# Autodesk Inventor assembly: CrossBot
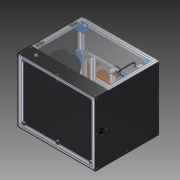
[picture p0: Inventor's stored thumbnail of the model, 180x180]
Saved by Autodesk Inventor 2015 SP1 (Build 190203100, 203)
## iProperties
Created: 2014-08-14
Part Number: CrossBot
Document SubType Name: Assembly
Designer: t_clevj
Mass: 14844.5 g
Surface Area: 49855.2 cm^2
Volume: 9320.22 cm^3
Density: 1.59271 g/cm^3
Author: t_clevj
## Documents named in this file (26)
- C:\Users\Jack\ownCloud\Projects\CrossBot\InventorModel\CrossBot.iam
- C:\Users\Jack\ownCloud\Projects\CrossBot\InventorModel\Frame\Frame.iam
- C:\Users\Jack\ownCloud\Projects\CrossBot\InventorModel\Hardware\Shaft\Shaft8\YShaft.ipt
- C:\Users\Jack\ownCloud\Projects\CrossBot\InventorModel\YAxis\YAxisMotorLeft.iam
- C:\Users\Jack\ownCloud\Projects\CrossBot\InventorModel\YAxis\YAxisIdlerLeft.iam
- C:\Users\Jack\ownCloud\Projects\CrossBot\InventorModel\YAxis\YAxisMotorRight.iam
- C:\Users\Jack\ownCloud\Projects\CrossBot\InventorModel\XAxis\XEndLeft.iam
- C:\Users\Jack\ownCloud\Projects\CrossBot\InventorModel\YAxis\YAxisIdlerRight.iam
- C:\Users\Jack\ownCloud\Projects\CrossBot\InventorModel\XAxis\XEndRight.iam
- C:\Users\Jack\ownCloud\Projects\CrossBot\InventorModel\Hardware\Shaft\Shaft8\XShaft.ipt
- C:\Users\Jack\ownCloud\Projects\CrossBot\InventorModel\Hardware\Shaft\Shaft10\ZAxisShaft.ipt
- C:\Users\Jack\ownCloud\Projects\CrossBot\InventorModel\Enclosure\SpoolFilament.ipt
- C:\Users\Jack\ownCloud\Projects\CrossBot\InventorModel\XAxis\XCarriage.iam
- C:\Users\Jack\ownCloud\Projects\CrossBot\InventorModel\Electronics\PSUUltibots.ipt
- C:\Users\Jack\ownCloud\Projects\CrossBot\InventorModel\Extruder\SanladererBowdenExtruder\SanladererBowdenExtruder.iam
- C:\Users\Jack\ownCloud\Projects\CrossBot\InventorModel\Extruder\SanladererBowdenExtruder\SanladererBowdenExtruderMirrored.iam
- C:\Users\Jack\ownCloud\Projects\CrossBot\InventorModel\ZAxis\ZAxisBed.iam
- C:\Users\Jack\ownCloud\Projects\CrossBot\InventorModel\Electronics\LCD\RepRapDiscountGLCD.ipt
- C:\Users\Jack\ownCloud\Projects\CrossBot\InventorModel\Electronics\Boards\Smoothieboard.ipt
- C:\Users\Jack\ownCloud\Projects\CrossBot\InventorModel\Hardware\Nuts\ExtrusionNuts\ExtrusionNutHNTT5-4.ipt
- C:\Users\Jack\ownCloud\Projects\CrossBot\InventorModel\ZAxis\ZAxisRodClamp.iam
- C:\Users\Jack\ownCloud\Projects\CrossBot\InventorModel\ZAxis\ZDrive.iam
- C:\Users\Jack\ownCloud\Projects\CrossBot\InventorModel\Electronics\KeySwitch\KeySwitch.iam
- C:\Users\Jack\ownCloud\Projects\CrossBot\InventorModel\Electronics\Fans\Fan40x20mm.ipt
- C:\Users\Jack\ownCloud\Projects\CrossBot\InventorModel\ZAxis\ZEndstop.iam
- C:\Users\Jack\ownCloud\Projects\CrossBot\InventorModel\Electronics\Ports\PowerSocket.ipt
## Components (63 placed, 25 different names)
1. Frame:1 [sub-assembly] — Mate:6, Mate:23, Mate:24, Mate:25, Mate:27, Mate:28, Mate:29, Mate:30, Mate:31, Mate:32, Mate:69, Mate:70, Angle:13, Angle:14, Mate:260, Flush:89, Mate:261, Flush:90, Angle:15, Mate:312, Mate:313, Mate:317, Angle:16, Mate:319, Angle:17, Mate:321, Angle:18, Mate:323, Angle:19, Mate:326, Mate:327, Angle:20, Angle:21, Mate:329, Angle:22, Mate:331, Angle:23, Mate:333, Angle:24, Mate:336, Angle:25, Mate:338, Angle:26, Mate:340, Angle:27, Mate:344, Angle:28, Mate:345, Angle:29, Flush:92, Flush:93, Flush:94, Flush:95, Mate:352, Mate:353, Mate:354, Mate:355, Flush:98, Mate:358, Angle:30, Mate:360, Angle:31, Mate:362, Angle:32, Mate:364, Angle:33, Mate:366, Angle:34, Mate:368, Mate:370, Angle:35, Mate:372, Angle:36, Angle:37, Mate:377, Mate:378, Mate:379, Mate:380, Angle:38, Angle:39, Angle:40, Angle:41, Mate:381, Mate:382, Mate:383, Angle:42, Angle:43, Angle:44, Angle:45, Mate:389, Mate:390, Mate:391, Mate:392, Mate:400, Mate:401, Mate:402, Angle:46, Mate:417, Mate:418, Mate:419, Mate:420, Mate:421, Mate:422, Mate:423, Mate:424, Mate:425, Mate:426, Mate:427, Mate:428
2. ZEndstop:1 [sub-assembly] — Mate:415, Angle:46, Mate:416
3. ZDrive:1 [sub-assembly] — Mate:381, Mate:382, Mate:383, Mate:384, Mate:385, Mate:386, Mate:387, Mate:388
4. ExtrusionNutHNTT5-4:29 — Mate:385, Angle:44, Mate:390
5. ExtrusionNutHNTT5-4:30 — Mate:386, Angle:45, Mate:389
6. ExtrusionNutHNTT5-4:31 — Mate:387, Angle:43, Mate:392
7. ExtrusionNutHNTT5-4:32 — Mate:388, Angle:42, Mate:391
8. ExtrusionNutHNTT5-4:16 — Mate:357, Mate:358, Angle:30
9. ExtrusionNutHNTT5-4:17 — Mate:359, Mate:360, Angle:31
10. ExtrusionNutHNTT5-4:18 — Mate:361, Mate:362, Angle:32
11. ExtrusionNutHNTT5-4:19 — Mate:363, Mate:364, Angle:33
12. ExtrusionNutHNTT5-4:20 — Mate:367, Angle:34, Mate:368
13. ExtrusionNutHNTT5-4:21 — Mate:365, Mate:366, Angle:37
14. ExtrusionNutHNTT5-4:22 — Mate:369, Mate:370, Angle:35
15. ExtrusionNutHNTT5-4:24 — Mate:371, Mate:372, Angle:36
16. ZAxisRodClamp:4 [sub-assembly] — Mate:350, Flush:95, Mate:355, Mate:365, Mate:367, Mate:384
17. ZAxisRodClamp:3 [sub-assembly] — Mate:349, Flush:94, Mate:352, Flush:97, Mate:357, Mate:359, Mate:416
18. ZAxisRodClamp:2 [sub-assembly] — Mate:348, Flush:92, Mate:354, Mate:369, Mate:371
19. ZAxisRodClamp:1 [sub-assembly] — Mate:347, Flush:93, Mate:353, Flush:96, Mate:361, Mate:363
20. ZAxisBed:1 [sub-assembly] — Mate:314, Mate:315
21. ZAxisShaft:1 — Mate:315, Mate:349, Mate:350, Mate:351, Flush:97, Mate:415
22. ZAxisShaft:2 — Mate:314, Mate:347, Mate:348, Mate:351, Flush:96
23. YShaft:2 — Mate:26, Mate:124, Mate:130, Mate:187
24. YShaft:3 — Mate:37, Mate:190
25. YAxisMotorLeft:1 [sub-assembly] — Mate:23, Mate:24, Mate:25, Mate:26, Mate:324, Mate:325, Mate:328, Mate:330
26. YAxisMotorRight:1 [sub-assembly] — Mate:30, Mate:31, Mate:32, Mate:37, Mate:316, Mate:318, Mate:320, Mate:322
27. YAxisIdlerLeft:1 [sub-assembly] — Mate:27, Mate:28, Mate:29, Mate:130, Mate:337, Mate:339, Mate:341
28. YAxisIdlerRight:1 [sub-assembly] — Mate:334, Mate:335, Mate:342, Mate:343, Mate:426, Mate:427, Mate:428
29. XShaft:1 — Mate:189, Flush:54, Mate:242
30. XShaft:2 — Mate:188, Flush:55, Mate:191, Mate:241
31. XCarriage:1 [sub-assembly] — Mate:241, Mate:242
32. XEndLeft:1 [sub-assembly] — Mate:124, Mate:187, Mate:188, Mate:189, Flush:54, Flush:55, Angle:14
33. XEndRight:1 [sub-assembly] — Mate:190, Mate:191, Angle:13
34. KeySwitch:1 [sub-assembly] — Mate:400, Mate:401, Mate:402
35. Fan40x20mm:1 — Mate:423, Mate:424, Mate:425
36. Fan40x20mm:3 — Mate:420, Mate:421, Mate:422
37. PowerSocket:1 — Mate:417, Mate:418, Mate:419
38. Smoothieboard:1 — Mate:312
39. RepRapDiscountGLCD:1 — Angle:15
40. PSUUltibots:1 — Mate:313
41. ExtrusionNutHNTT5-4:25 — Mate:373, Mate:380, Angle:38
42. ExtrusionNutHNTT5-4:26 — Mate:374, Mate:378, Angle:39
43. ExtrusionNutHNTT5-4:27 — Mate:375, Mate:379, Angle:40
44. ExtrusionNutHNTT5-4:28 — Mate:376, Mate:377, Angle:41
45. SanladererBowdenExtruderMirrored:1 [sub-assembly] — Mate:261, Flush:90, Flush:91, Mate:373, Mate:376
46. SanladererBowdenExtruder:1 [sub-assembly] — Mate:260, Flush:89, Flush:91, Flush:98, Mate:374, Mate:375
47. SpoolFilament:2 — Mate:309
48. SpoolFilament:1 — Mate:309
49. ExtrusionNutHNTT5-4:1 — Mate:316, Mate:317, Angle:16
50. ExtrusionNutHNTT5-4:2 — Mate:318, Mate:319, Angle:17
51. ExtrusionNutHNTT5-4:3 — Mate:320, Mate:321, Angle:18
52. ExtrusionNutHNTT5-4:4 — Mate:322, Mate:323, Angle:19
53. ExtrusionNutHNTT5-4:5 — Mate:324, Mate:327, Angle:20
54. ExtrusionNutHNTT5-4:6 — Mate:325, Mate:326, Angle:21
55. ExtrusionNutHNTT5-4:7 — Mate:328, Mate:329, Angle:22
56. ExtrusionNutHNTT5-4:8 — Mate:330, Mate:331, Angle:23
57. ExtrusionNutHNTT5-4:9 — Mate:333, Angle:24, Mate:334
58. ExtrusionNutHNTT5-4:10 — Mate:335, Mate:336, Angle:25
59. ExtrusionNutHNTT5-4:11 — Mate:337, Mate:338, Angle:26
60. ExtrusionNutHNTT5-4:12 — Mate:339, Mate:340, Angle:27
61. ExtrusionNutHNTT5-4:13 — Mate:341, Mate:345, Angle:29
62. ExtrusionNutHNTT5-4:14 — Mate:342
63. ExtrusionNutHNTT5-4:15 — Mate:343, Mate:344, Angle:28
## Relationships (167: Mate 121, Angle 34, Flush 12)
- Mate:6: Frame:1
- Mate:23: Frame:1 ↔ YAxisMotorLeft:1
- Mate:24: Frame:1 ↔ YAxisMotorLeft:1
- Mate:25: Frame:1 ↔ YAxisMotorLeft:1
- Mate:26: YShaft:2 ↔ YAxisMotorLeft:1
- Mate:27: Frame:1 ↔ YAxisIdlerLeft:1
- Mate:28: Frame:1 ↔ YAxisIdlerLeft:1
- Mate:29: Frame:1 ↔ YAxisIdlerLeft:1
- Mate:30: Frame:1 ↔ YAxisMotorRight:1
- Mate:31: Frame:1 ↔ YAxisMotorRight:1
- Mate:32: Frame:1 ↔ YAxisMotorRight:1
- Mate:37: YShaft:3 ↔ YAxisMotorRight:1
- Mate:69: Frame:1
- Mate:70: Frame:1
- Mate:124: YShaft:2 ↔ XEndLeft:1
- Mate:130: YShaft:2 ↔ YAxisIdlerLeft:1
- Mate:187: YShaft:2 ↔ XEndLeft:1
- Mate:188: XShaft:2 ↔ XEndLeft:1
- Mate:189: XShaft:1 ↔ XEndLeft:1
- Flush:54: XShaft:1 ↔ XEndLeft:1
- Flush:55: XShaft:2 ↔ XEndLeft:1
- Mate:190: YShaft:3 ↔ XEndRight:1
- Mate:191: XShaft:2 ↔ XEndRight:1
- Angle:13 (0 deg): Frame:1 ↔ XEndRight:1
- Angle:14 (0 deg): Frame:1 ↔ XEndLeft:1
- Mate:241: XShaft:2 ↔ XCarriage:1
- Mate:242: XShaft:1 ↔ XCarriage:1
- Mate:260: Frame:1 ↔ SanladererBowdenExtruder:1
- Flush:89 (2 mm): Frame:1 ↔ SanladererBowdenExtruder:1
- Mate:261: Frame:1 ↔ SanladererBowdenExtruderMirrored:1
- Flush:90 (2 mm): Frame:1 ↔ SanladererBowdenExtruderMirrored:1
- Flush:91: SanladererBowdenExtruderMirrored:1 ↔ SanladererBowdenExtruder:1
- Angle:15 (60 deg): Frame:1 ↔ RepRapDiscountGLCD:1
- Mate:309: SpoolFilament:2 ↔ SpoolFilament:1
- Mate:312 (15 mm): Frame:1 ↔ Smoothieboard:1
- Mate:313: Frame:1 ↔ PSUUltibots:1
- Mate:314: ZAxisBed:1 ↔ ZAxisShaft:2
- Mate:315: ZAxisBed:1 ↔ ZAxisShaft:1
- Mate:316: YAxisMotorRight:1 ↔ ExtrusionNutHNTT5-4:1
- Mate:317: Frame:1 ↔ ExtrusionNutHNTT5-4:1
- Angle:16 (0 deg): Frame:1 ↔ ExtrusionNutHNTT5-4:1
- Mate:318: YAxisMotorRight:1 ↔ ExtrusionNutHNTT5-4:2
- Mate:319: Frame:1 ↔ ExtrusionNutHNTT5-4:2
- Angle:17 (0 deg): Frame:1 ↔ ExtrusionNutHNTT5-4:2
- Mate:320: YAxisMotorRight:1 ↔ ExtrusionNutHNTT5-4:3
- Mate:321: Frame:1 ↔ ExtrusionNutHNTT5-4:3
- Angle:18 (0 deg): Frame:1 ↔ ExtrusionNutHNTT5-4:3
- Mate:322: YAxisMotorRight:1 ↔ ExtrusionNutHNTT5-4:4
- Mate:323: Frame:1 ↔ ExtrusionNutHNTT5-4:4
- Angle:19 (0 deg): Frame:1 ↔ ExtrusionNutHNTT5-4:4
- Mate:324: YAxisMotorLeft:1 ↔ ExtrusionNutHNTT5-4:5
- Mate:325: YAxisMotorLeft:1 ↔ ExtrusionNutHNTT5-4:6
- Mate:326: Frame:1 ↔ ExtrusionNutHNTT5-4:6
- Mate:327: Frame:1 ↔ ExtrusionNutHNTT5-4:5
- Angle:20 (0 deg): Frame:1 ↔ ExtrusionNutHNTT5-4:5
- Angle:21 (0 deg): Frame:1 ↔ ExtrusionNutHNTT5-4:6
- Mate:328: YAxisMotorLeft:1 ↔ ExtrusionNutHNTT5-4:7
- Mate:329: Frame:1 ↔ ExtrusionNutHNTT5-4:7
- Angle:22 (0 deg): Frame:1 ↔ ExtrusionNutHNTT5-4:7
- Mate:330: YAxisMotorLeft:1 ↔ ExtrusionNutHNTT5-4:8
- Mate:331: Frame:1 ↔ ExtrusionNutHNTT5-4:8
- Angle:23 (0 deg): Frame:1 ↔ ExtrusionNutHNTT5-4:8
- Mate:333: Frame:1 ↔ ExtrusionNutHNTT5-4:9
- Angle:24 (0 deg): Frame:1 ↔ ExtrusionNutHNTT5-4:9
- Mate:334: YAxisIdlerRight:1 ↔ ExtrusionNutHNTT5-4:9
- Mate:335: YAxisIdlerRight:1 ↔ ExtrusionNutHNTT5-4:10
- Mate:336: Frame:1 ↔ ExtrusionNutHNTT5-4:10
- Angle:25 (0 deg): Frame:1 ↔ ExtrusionNutHNTT5-4:10
- Mate:337: YAxisIdlerLeft:1 ↔ ExtrusionNutHNTT5-4:11
- Mate:338: Frame:1 ↔ ExtrusionNutHNTT5-4:11
- Angle:26 (0 deg): Frame:1 ↔ ExtrusionNutHNTT5-4:11
- Mate:339: YAxisIdlerLeft:1 ↔ ExtrusionNutHNTT5-4:12
- Mate:340: Frame:1 ↔ ExtrusionNutHNTT5-4:12
- Angle:27 (0 deg): Frame:1 ↔ ExtrusionNutHNTT5-4:12
- Mate:341: YAxisIdlerLeft:1 ↔ ExtrusionNutHNTT5-4:13
- Mate:342: YAxisIdlerRight:1 ↔ ExtrusionNutHNTT5-4:14
- Mate:343: YAxisIdlerRight:1 ↔ ExtrusionNutHNTT5-4:15
- Mate:344: Frame:1 ↔ ExtrusionNutHNTT5-4:15
- Angle:28 (0 deg): Frame:1 ↔ ExtrusionNutHNTT5-4:15
- Mate:345: Frame:1 ↔ ExtrusionNutHNTT5-4:13
- Angle:29 (0 deg): Frame:1 ↔ ExtrusionNutHNTT5-4:13
- Mate:347: ZAxisRodClamp:1 ↔ ZAxisShaft:2
- Mate:348: ZAxisRodClamp:2 ↔ ZAxisShaft:2
- Flush:92: Frame:1 ↔ ZAxisRodClamp:2
- Flush:93: Frame:1 ↔ ZAxisRodClamp:1
- Mate:349: ZAxisRodClamp:3 ↔ ZAxisShaft:1
- Flush:94: Frame:1 ↔ ZAxisRodClamp:3
- Mate:350: ZAxisRodClamp:4 ↔ ZAxisShaft:1
- Flush:95: Frame:1 ↔ ZAxisRodClamp:4
- Mate:351 (130 mm): ZAxisShaft:1 ↔ ZAxisShaft:2
- Mate:352: Frame:1 ↔ ZAxisRodClamp:3
- Mate:353: Frame:1 ↔ ZAxisRodClamp:1
- Mate:354: Frame:1 ↔ ZAxisRodClamp:2
- Mate:355: Frame:1 ↔ ZAxisRodClamp:4
- Flush:96: ZAxisRodClamp:1 ↔ ZAxisShaft:2
- Flush:97: ZAxisRodClamp:3 ↔ ZAxisShaft:1
- Flush:98 (82 mm): Frame:1 ↔ SanladererBowdenExtruder:1
- Mate:357: ExtrusionNutHNTT5-4:16 ↔ ZAxisRodClamp:3
- Mate:358: Frame:1 ↔ ExtrusionNutHNTT5-4:16
- Angle:30 (0 deg): Frame:1 ↔ ExtrusionNutHNTT5-4:16
- Mate:359: ExtrusionNutHNTT5-4:17 ↔ ZAxisRodClamp:3
- Mate:360: Frame:1 ↔ ExtrusionNutHNTT5-4:17
- Angle:31 (0 deg): Frame:1 ↔ ExtrusionNutHNTT5-4:17
- Mate:361: ExtrusionNutHNTT5-4:18 ↔ ZAxisRodClamp:1
- Mate:362: Frame:1 ↔ ExtrusionNutHNTT5-4:18
- Angle:32 (0 deg): Frame:1 ↔ ExtrusionNutHNTT5-4:18
- Mate:363: ExtrusionNutHNTT5-4:19 ↔ ZAxisRodClamp:1
- Mate:364: Frame:1 ↔ ExtrusionNutHNTT5-4:19
- Angle:33 (0 deg): Frame:1 ↔ ExtrusionNutHNTT5-4:19
- Mate:365: ExtrusionNutHNTT5-4:21 ↔ ZAxisRodClamp:4
- Mate:366: Frame:1 ↔ ExtrusionNutHNTT5-4:21
- Mate:367: ExtrusionNutHNTT5-4:20 ↔ ZAxisRodClamp:4
- Angle:34 (0 deg): Frame:1 ↔ ExtrusionNutHNTT5-4:20
- Mate:368: Frame:1 ↔ ExtrusionNutHNTT5-4:20
- Mate:369: ExtrusionNutHNTT5-4:22 ↔ ZAxisRodClamp:2
- Mate:370: Frame:1 ↔ ExtrusionNutHNTT5-4:22
- Angle:35 (0 deg): Frame:1 ↔ ExtrusionNutHNTT5-4:22
- Mate:371: ExtrusionNutHNTT5-4:24 ↔ ZAxisRodClamp:2
- Mate:372: Frame:1 ↔ ExtrusionNutHNTT5-4:24
- Angle:36 (0 deg): Frame:1 ↔ ExtrusionNutHNTT5-4:24
- Angle:37 (0 deg): Frame:1 ↔ ExtrusionNutHNTT5-4:21
- Mate:373: ExtrusionNutHNTT5-4:25 ↔ SanladererBowdenExtruderMirrored:1
- Mate:374: ExtrusionNutHNTT5-4:26 ↔ SanladererBowdenExtruder:1
- Mate:375: ExtrusionNutHNTT5-4:27 ↔ SanladererBowdenExtruder:1
- Mate:376: ExtrusionNutHNTT5-4:28 ↔ SanladererBowdenExtruderMirrored:1
- Mate:377: Frame:1 ↔ ExtrusionNutHNTT5-4:28
- Mate:378: Frame:1 ↔ ExtrusionNutHNTT5-4:26
- Mate:379: Frame:1 ↔ ExtrusionNutHNTT5-4:27
- Mate:380: Frame:1 ↔ ExtrusionNutHNTT5-4:25
- Angle:38 (0 deg): Frame:1 ↔ ExtrusionNutHNTT5-4:25
- Angle:39 (0 deg): Frame:1 ↔ ExtrusionNutHNTT5-4:26
- Angle:40 (0 deg): Frame:1 ↔ ExtrusionNutHNTT5-4:27
- Angle:41 (0 deg): Frame:1 ↔ ExtrusionNutHNTT5-4:28
- Mate:381: Frame:1 ↔ ZDrive:1
- Mate:382: Frame:1 ↔ ZDrive:1
- Mate:383 (205 mm): Frame:1 ↔ ZDrive:1
- Mate:384 (24.5 mm): ZDrive:1 ↔ ZAxisRodClamp:4
- Mate:385: ZDrive:1 ↔ ExtrusionNutHNTT5-4:29
- Mate:386: ZDrive:1 ↔ ExtrusionNutHNTT5-4:30
- Mate:387: ZDrive:1 ↔ ExtrusionNutHNTT5-4:31
- Mate:388: ZDrive:1 ↔ ExtrusionNutHNTT5-4:32
- Angle:42 (0 deg): Frame:1 ↔ ExtrusionNutHNTT5-4:32
- Angle:43 (0 deg): Frame:1 ↔ ExtrusionNutHNTT5-4:31
- Angle:44 (0 deg): Frame:1 ↔ ExtrusionNutHNTT5-4:29
- Angle:45 (0 deg): Frame:1 ↔ ExtrusionNutHNTT5-4:30
- Mate:389: Frame:1 ↔ ExtrusionNutHNTT5-4:30
- Mate:390: Frame:1 ↔ ExtrusionNutHNTT5-4:29
- Mate:391: Frame:1 ↔ ExtrusionNutHNTT5-4:32
- Mate:392: Frame:1 ↔ ExtrusionNutHNTT5-4:31
- Mate:400: Frame:1 ↔ KeySwitch:1
- Mate:401: Frame:1 ↔ KeySwitch:1
- Mate:402: Frame:1 ↔ KeySwitch:1
- Mate:415: ZEndstop:1 ↔ ZAxisShaft:1
- Angle:46 (0 deg): Frame:1 ↔ ZEndstop:1
- Mate:416 (6.5 mm): ZEndstop:1 ↔ ZAxisRodClamp:3
- Mate:417: Frame:1 ↔ PowerSocket:1
- Mate:418: Frame:1 ↔ PowerSocket:1
- Mate:419: Frame:1 ↔ PowerSocket:1
- Mate:420: Frame:1 ↔ Fan40x20mm:3
- Mate:421: Frame:1 ↔ Fan40x20mm:3
- Mate:422: Frame:1 ↔ Fan40x20mm:3
- Mate:423: Frame:1 ↔ Fan40x20mm:1
- Mate:424: Frame:1 ↔ Fan40x20mm:1
- Mate:425: Frame:1 ↔ Fan40x20mm:1
- Mate:426: Frame:1 ↔ YAxisIdlerRight:1
- Mate:427: Frame:1 ↔ YAxisIdlerRight:1
- Mate:428: Frame:1 ↔ YAxisIdlerRight:1
